# Autodesk Inventor assembly: Blue Alliance Bucket
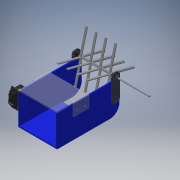
[picture p0: Inventor's stored thumbnail of the model, 180x180]
Saved by Autodesk Inventor 2016 (Build 200138000, 138)
## iProperties
Created: 2015-12-16
Part Number: Blue Alliance Bucket
Document SubType Name: Assembly
Designer: TimB
Author: TimB
## Documents named in this file (11)
- C:\Users\TimB\Documents\GitHub\phi_robotics\3d-models\FTC_Tetrix_KOP_Block_Party\Tim Bloot Designs\JAr JaR Bot\Blue Alliance Bucket.iam
- C:\Users\TimB\Documents\GitHub\phi_robotics\3d-models\FTC_Tetrix_KOP_Block_Party\Tim Bloot Designs\JAr JaR Bot\Bucket - BlueA.ipt
- C:\Users\TimB\Documents\GitHub\phi_robotics\3d-models\FTC_Tetrix_KOP_Block_Party\Tetrix_Kit_FTC\Autodesk Inventor Files\tetrix_servo_mount.ipt
- C:\Users\TimB\Documents\GitHub\phi_robotics\3d-models\FTC_Tetrix_KOP_Block_Party\Tetrix_Kit_FTC\Autodesk Inventor Files\tetrix_739061_2012.ipt
- C:\Users\TimB\Documents\GitHub\phi_robotics\3d-models\FTC_Tetrix_KOP_Block_Party\Tim Bloot Designs\JAr JaR Bot\Bucket -  Top.ipt
- C:\Users\TimB\Documents\GitHub\phi_robotics\3d-models\FTC_Tetrix_KOP_Block_Party\Tetrix_Kit_FTC\Autodesk Inventor Files\tetrix_servo_body.ipt
- C:\Users\TimB\Documents\GitHub\phi_robotics\3d-models\FTC_Tetrix_KOP_Block_Party\Tetrix_Kit_FTC\Autodesk Inventor Files\tetrix_axle-long.ipt
- C:\Users\TimB\Documents\GitHub\phi_robotics\3d-models\FTC_Tetrix_KOP_Block_Party\Tetrix_Kit_FTC\Autodesk Inventor Files\tetrix_739092_2012.iam
- C:\Users\TimB\Documents\GitHub\phi_robotics\3d-models\FTC_Tetrix_KOP_Block_Party\Tetrix_Kit_FTC\Autodesk Inventor Files\tetrix_bushing.ipt
- C:\Users\TimB\Documents\GitHub\phi_robotics\3d-models\FTC_Tetrix_KOP_Block_Party\Tim Bloot Designs\JAr JaR Bot\Bucket - Rake.ipt
- C:\Users\TimB\Documents\GitHub\phi_robotics\3d-models\FTC_Tetrix_KOP_Block_Party\Tim Bloot Designs\JAr JaR Bot\Bucket - 4 Rake.iam
## Components (13 placed, 10 different names)
1. Bucket - BlueA:1 — Rigid:1, Rigid:2, Rigid:3, Rigid:4
2. tetrix_servo_mount:1 — Rigid:1, Rigid:5
3. tetrix_739061_2012:1 — Rigid:2, Rotational:3
4. tetrix_739061_2012:2 — Rigid:3, Rotational:4
5. Bucket -  Top:1 — Rigid:4
6. tetrix_servo_body:1 — Rigid:5
7. tetrix_axle-long:1 — Rigid:6, Rigid:7, Rigid:8, Rigid:9
8. tetrix_739092_2012:1 [sub-assembly] — Rigid:7
9. tetrix_739092_2012:2 [sub-assembly] — Rigid:6, Rotational:5
10. tetrix_bushing:1 — Rotational:3
11. Bucket - Rake:1 — Rigid:8
12. Bucket - 4 Rake:1 [sub-assembly] — Rigid:9
13. tetrix_bushing:2 — Rotational:4, Rotational:5
## Relationships (12: WeldJoint 9, RevoluteJoint 3)
- Rigid:1 [WeldJoint]: Bucket - BlueA:1 ↔ tetrix_servo_mount:1
- Rigid:2 [WeldJoint]: Bucket - BlueA:1 ↔ tetrix_739061_2012:1
- Rigid:3 [WeldJoint]: Bucket - BlueA:1 ↔ tetrix_739061_2012:2
- Rigid:4 [WeldJoint]: Bucket - BlueA:1 ↔ Bucket -  Top:1
- Rigid:5 [WeldJoint]: tetrix_servo_mount:1 ↔ tetrix_servo_body:1
- Rigid:6 [WeldJoint]: tetrix_axle-long:1 ↔ tetrix_739092_2012:2
- Rotational:3 [RevoluteJoint]: tetrix_739061_2012:1 ↔ tetrix_bushing:1
- Rigid:7 [WeldJoint] (-109.601 mm): tetrix_axle-long:1 ↔ tetrix_739092_2012:1
- Rigid:8 [WeldJoint] (-10.16 mm): tetrix_axle-long:1 ↔ Bucket - Rake:1
- Rigid:9 [WeldJoint] (-8.89 mm): tetrix_axle-long:1 ↔ Bucket - 4 Rake:1
- Rotational:4 [RevoluteJoint]: tetrix_739061_2012:2 ↔ tetrix_bushing:2
- Rotational:5 [RevoluteJoint]: tetrix_739092_2012:2 ↔ tetrix_bushing:2
